# Autodesk Inventor assembly: ORBD Assembly
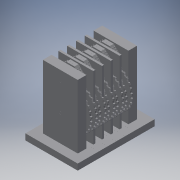
[picture p0: Inventor's stored thumbnail of the model, 180x180]
Saved by Autodesk Inventor 2017 (Build 210142000, 142)
## iProperties
Created: 2018-03-04
Part Number: ORBD Assembly
Document SubType Name: Assembly
Designer: Russ
Author: Russ
## Documents named in this file (7)
- C:\Users\Russ\Desktop\3D Models\ORBD\ORBD Assembly.iam
- C:\Users\Russ\Desktop\3D Models\ORBD\Left Braille Wheel.ipt
- C:\Users\Russ\Desktop\3D Models\ORBD\Middle Gear.ipt
- C:\Users\Russ\Desktop\3D Models\ORBD\End Frame.ipt
- C:\Users\Russ\Desktop\3D Models\ORBD\Axle.ipt
- C:\Users\Russ\Desktop\3D Models\ORBD\Middle Frame.ipt
- C:\Users\Russ\Desktop\3D Models\ORBD\Right Braille Wheel.ipt
## Components (28 placed, 6 different names)
1. End Frame:1 — Mate:3, Mate:4, Mate:5, Mate:6, Flush:2, Flush:3, Mate:7, Mate:8, Angle:1, Flush:6, Flush:7, Angle:5, Flush:16
2. Left Braille Wheel:1 — Mate:1, Mate:5, Mate:6, Rotation:1, Angle:1, Mate:16
3. Middle Gear:1 — Mate:1, Mate:3, Mate:4, Rotation:1
4. Right Braille Wheel:1 — Mate:15, Mate:16, Angle:5, Rotation:2
5. Middle Gear:2 — Mate:12, Rotation:2
6. Axle:1 — Flush:3, Mate:8, Mate:12, Mate:19, Mate:23, Mate:28, Mate:32, Mate:37, Mate:44, Mate:46, Mate:50
7. Axle:2 — Flush:2, Mate:7, Mate:15, Mate:17, Mate:21, Mate:26, Mate:30, Mate:35, Mate:36, Mate:38, Mate:39
8. Middle Frame:1 — Flush:6, Flush:7, Mate:18, Mate:20, Mate:25, Flush:10, Flush:11, Angle:6, Angle:7
9. Left Braille Wheel:2 — Mate:17, Mate:18, Mate:22, Angle:6, Rotation:3
10. Middle Gear:3 — Mate:19, Mate:20, Rotation:3
11. Middle Gear:4 — Mate:23, Mate:24, Rotation:4
12. Right Braille Wheel:2 — Mate:21, Mate:22, Mate:24, Angle:7, Rotation:4
13. Right Braille Wheel:3 — Mate:30, Mate:31, Mate:33, Angle:9, Rotation:6
14. Right Braille Wheel:4 — Mate:36, Mate:41, Angle:11, Rotation:8
15. Right Braille Wheel:5 — Mate:39, Mate:49, Mate:51, Angle:13, Rotation:10
16. Middle Gear:5 — Mate:28, Mate:29, Rotation:5
17. Middle Gear:6 — Mate:32, Mate:33, Rotation:6
18. Middle Gear:7 — Mate:37, Mate:42, Rotation:7
19. Left Braille Wheel:3 — Mate:26, Mate:27, Mate:31, Angle:8, Rotation:5
20. Left Braille Wheel:4 — Mate:35, Mate:40, Mate:41, Angle:10, Rotation:7
21. Left Braille Wheel:5 — Mate:38, Mate:48, Mate:49, Angle:12, Rotation:9
22. Middle Frame:2 — Mate:25, Flush:10, Flush:11, Mate:27, Mate:29, Mate:34, Flush:12, Flush:13, Angle:8, Angle:9
23. Middle Frame:3 — Mate:34, Flush:12, Flush:13, Mate:40, Mate:42, Mate:43, Flush:14, Flush:15, Flush:17, Angle:10, Angle:11
24. Middle Frame:4 — Mate:43, Flush:14, Flush:15, Mate:45, Mate:47, Mate:48, Mate:52, Angle:12, Angle:13
25. End Frame:2 — Mate:52, Flush:16, Flush:17
26. Middle Gear:8 — Mate:44, Mate:45, Rotation:8
27. Middle Gear:9 — Mate:46, Mate:47, Rotation:9
28. Middle Gear:10 — Mate:50, Mate:51, Rotation:10
## Relationships (78: Mate 46, Flush 12, RelateRotation 10, Angle 10)
- Mate:1: Left Braille Wheel:1 ↔ Middle Gear:1
- Mate:3: End Frame:1 ↔ Middle Gear:1
- Mate:4: End Frame:1 ↔ Middle Gear:1
- Mate:5: End Frame:1 ↔ Left Braille Wheel:1
- Mate:6: End Frame:1 ↔ Left Braille Wheel:1
- Flush:2: End Frame:1 ↔ Axle:2
- Flush:3: End Frame:1 ↔ Axle:1
- Mate:7: End Frame:1 ↔ Axle:2
- Mate:8: End Frame:1 ↔ Axle:1
- Rotation:1 [RelateRotation] (4 ul): Left Braille Wheel:1 ↔ Middle Gear:1
- Mate:12: Middle Gear:2 ↔ Axle:1
- Angle:1 (0 deg): End Frame:1 ↔ Left Braille Wheel:1
- Flush:6: End Frame:1 ↔ Middle Frame:1
- Flush:7: End Frame:1 ↔ Middle Frame:1
- Mate:15: Right Braille Wheel:1 ↔ Axle:2
- Mate:16: Left Braille Wheel:1 ↔ Right Braille Wheel:1
- Angle:5 (0 deg): End Frame:1 ↔ Right Braille Wheel:1
- Rotation:2 [RelateRotation] (4 ul): Right Braille Wheel:1 ↔ Middle Gear:2
- Mate:17: Axle:2 ↔ Left Braille Wheel:2
- Mate:18: Middle Frame:1 ↔ Left Braille Wheel:2
- Mate:19: Axle:1 ↔ Middle Gear:3
- Mate:20: Middle Frame:1 ↔ Middle Gear:3
- Mate:21: Axle:2 ↔ Right Braille Wheel:2
- Mate:22: Left Braille Wheel:2 ↔ Right Braille Wheel:2
- Mate:23: Axle:1 ↔ Middle Gear:4
- Mate:24: Middle Gear:4 ↔ Right Braille Wheel:2
- Mate:25: Middle Frame:1 ↔ Middle Frame:2
- Flush:10: Middle Frame:1 ↔ Middle Frame:2
- Flush:11: Middle Frame:1 ↔ Middle Frame:2
- Mate:26: Axle:2 ↔ Left Braille Wheel:3
- Mate:27: Left Braille Wheel:3 ↔ Middle Frame:2
- Mate:28: Axle:1 ↔ Middle Gear:5
- Mate:29: Middle Gear:5 ↔ Middle Frame:2
- Mate:30: Axle:2 ↔ Right Braille Wheel:3
- Mate:31: Right Braille Wheel:3 ↔ Left Braille Wheel:3
- Mate:32: Axle:1 ↔ Middle Gear:6
- Mate:33: Right Braille Wheel:3 ↔ Middle Gear:6
- Mate:34: Middle Frame:2 ↔ Middle Frame:3
- Flush:12: Middle Frame:2 ↔ Middle Frame:3
- Flush:13: Middle Frame:2 ↔ Middle Frame:3
- Mate:35: Axle:2 ↔ Left Braille Wheel:4
- Mate:36: Axle:2 ↔ Right Braille Wheel:4
- Mate:37: Axle:1 ↔ Middle Gear:7
- Mate:38: Axle:2 ↔ Left Braille Wheel:5
- Mate:39: Axle:2 ↔ Right Braille Wheel:5
- Mate:40: Left Braille Wheel:4 ↔ Middle Frame:3
- Mate:41: Right Braille Wheel:4 ↔ Left Braille Wheel:4
- Mate:42: Middle Gear:7 ↔ Middle Frame:3
- Mate:43: Middle Frame:3 ↔ Middle Frame:4
- Flush:14: Middle Frame:3 ↔ Middle Frame:4
- Flush:15: Middle Frame:3 ↔ Middle Frame:4
- Mate:44: Axle:1 ↔ Middle Gear:8
- Mate:45: Middle Frame:4 ↔ Middle Gear:8
- Mate:46: Axle:1 ↔ Middle Gear:9
- Mate:47: Middle Frame:4 ↔ Middle Gear:9
- Mate:48: Left Braille Wheel:5 ↔ Middle Frame:4
- Mate:49: Right Braille Wheel:5 ↔ Left Braille Wheel:5
- Mate:50: Axle:1 ↔ Middle Gear:10
- Mate:51: Right Braille Wheel:5 ↔ Middle Gear:10
- Mate:52: Middle Frame:4 ↔ End Frame:2
- Flush:16: End Frame:1 ↔ End Frame:2
- Flush:17: Middle Frame:3 ↔ End Frame:2
- Angle:6 (0 deg): Middle Frame:1 ↔ Left Braille Wheel:2
- Angle:7 (0 deg): Middle Frame:1 ↔ Right Braille Wheel:2
- Angle:8 (0 deg): Left Braille Wheel:3 ↔ Middle Frame:2
- Angle:9 (0 deg): Right Braille Wheel:3 ↔ Middle Frame:2
- Angle:10 (0 deg): Left Braille Wheel:4 ↔ Middle Frame:3
- Angle:11 (0 deg): Right Braille Wheel:4 ↔ Middle Frame:3
- Angle:12 (0 deg): Left Braille Wheel:5 ↔ Middle Frame:4
- Angle:13 (0 deg): Right Braille Wheel:5 ↔ Middle Frame:4
- Rotation:3 [RelateRotation] (4 ul): Left Braille Wheel:2 ↔ Middle Gear:3
- Rotation:4 [RelateRotation] (4 ul): Middle Gear:4 ↔ Right Braille Wheel:2
- Rotation:5 [RelateRotation] (4 ul): Middle Gear:5 ↔ Left Braille Wheel:3
- Rotation:6 [RelateRotation] (4 ul): Right Braille Wheel:3 ↔ Middle Gear:6
- Rotation:7 [RelateRotation] (4 ul): Middle Gear:7 ↔ Left Braille Wheel:4
- Rotation:8 [RelateRotation] (4 ul): Right Braille Wheel:4 ↔ Middle Gear:8
- Rotation:9 [RelateRotation] (4 ul): Left Braille Wheel:5 ↔ Middle Gear:9
- Rotation:10 [RelateRotation] (4 ul): Right Braille Wheel:5 ↔ Middle Gear:10
